# Autodesk Inventor assembly: Slide rod assembly
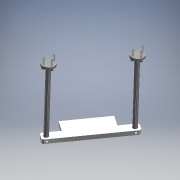
[picture p0: Inventor's stored thumbnail of the model, 180x180]
Saved by Autodesk Inventor 2017 (Build 210142000, 142)
## iProperties
Created: 2016-12-06
Part Number: Slide rod assembly
Document SubType Name: Assembly
Designer: qupec
Author: qupec
## Documents named in this file (4)
- C:\UMD\BPP\ROCKSAT X\STAR\CAD\Mechanical\Full payload assembly\Subsystems\Slide Rods\Slide rod assembly.iam
- C:\UMD\BPP\ROCKSAT X\STAR\CAD\Mechanical\Full payload assembly\Subsystems\Slide Rods\Slide rod connector.ipt
- C:\UMD\BPP\ROCKSAT X\STAR\CAD\Mechanical\Full payload assembly\Subsystems\Slide Rods\slide rod.ipt
- C:\UMD\BPP\ROCKSAT X\STAR\CAD\Mechanical\Full payload assembly\Subsystems\Fasteners\4-40 .5in Socket Screw.ipt
## Components (9 placed, 3 different names)
1. Slide rod connector:1 — Mate:1, Flush:1, Flush:2, Mate:18
2. slide rod:1 — Flush:2, Mate:18, Mate:22, Mate:23, Mate:24, Mate:25, Mate:26, Mate:27
3. slide rod:2 — Mate:1, Flush:1, Mate:19, Mate:20, Mate:21, Mate:28, Mate:29, Mate:30
4. 4-40 .5in Socket Screw:1 — Mate:23, Mate:27
5. 4-40 .5in Socket Screw:2 — Mate:24, Mate:26
6. 4-40 .5in Socket Screw:3 — Mate:22, Mate:25
7. 4-40 .5in Socket Screw:4 — Mate:21, Mate:29
8. 4-40 .5in Socket Screw:5 — Mate:20, Mate:28
9. 4-40 .5in Socket Screw:6 — Mate:19, Mate:30
## Relationships (16: Mate 14, Flush 2)
- Mate:1: Slide rod connector:1 ↔ slide rod:2
- Flush:1: Slide rod connector:1 ↔ slide rod:2
- Flush:2: Slide rod connector:1 ↔ slide rod:1
- Mate:18: Slide rod connector:1 ↔ slide rod:1
- Mate:19: slide rod:2 ↔ 4-40 .5in Socket Screw:6
- Mate:20: slide rod:2 ↔ 4-40 .5in Socket Screw:5
- Mate:21: slide rod:2 ↔ 4-40 .5in Socket Screw:4
- Mate:22: slide rod:1 ↔ 4-40 .5in Socket Screw:3
- Mate:23: slide rod:1 ↔ 4-40 .5in Socket Screw:1
- Mate:24: slide rod:1 ↔ 4-40 .5in Socket Screw:2
- Mate:25: slide rod:1 ↔ 4-40 .5in Socket Screw:3
- Mate:26: slide rod:1 ↔ 4-40 .5in Socket Screw:2
- Mate:27: slide rod:1 ↔ 4-40 .5in Socket Screw:1
- Mate:28: slide rod:2 ↔ 4-40 .5in Socket Screw:5
- Mate:29: slide rod:2 ↔ 4-40 .5in Socket Screw:4
- Mate:30: slide rod:2 ↔ 4-40 .5in Socket Screw:6
